# Autodesk Inventor assembly: 組合2
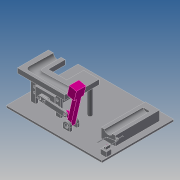
[picture p0: Inventor's stored thumbnail of the model, 180x180]
Saved by Autodesk Inventor 2015 (Build 190159000, 159)
## iProperties
Created: 2017-12-26
Part Number: 組合2
Document SubType Name: Assembly
Designer: user
Author: user
## Documents named in this file (7)
- C:\Users\user\Desktop\電腦輔助設計\組合2.iam
- C:\Users\user\Desktop\電腦輔助設計\01底板.ipt
- C:\Users\user\Desktop\電腦輔助設計\02連桿25.ipt
- C:\Users\user\Desktop\電腦輔助設計\03連桿15.ipt
- C:\Users\user\Desktop\電腦輔助設計\馬達.ipt
- C:\Users\user\Desktop\電腦輔助設計\連趕2.ipt
- C:\Users\user\Desktop\電腦輔助設計\槓桿.ipt
## Components (7 placed, 6 different names)
1. 01底板:1 — 插入:1, 貼合:1, 插入:4, 貼合:4, 角度:1, 插入:5
2. 02連桿25:1 — 插入:3, 貼合:3
3. 03連桿15:1 — 貼合:2, 插入:2, 插入:3, 角度:1
4. 馬達:1 — 插入:1, 貼合:1, 貼合:2
5. 連趕2:1 — 插入:4, 貼合:5
6. 02連桿25:2 — 插入:2, 貼合:3, 貼合:4, 貼合:5
7. 槓桿:2 — 插入:5
## Relationships (11: Insert 5, Mate 5, Angle 1)
- 插入:1 [Insert]: 01底板:1 ↔ 馬達:1
- 貼合:1 [Mate]: 01底板:1 ↔ 馬達:1
- 貼合:2 [Mate]: 03連桿15:1 ↔ 馬達:1
- 插入:2 [Insert]: 03連桿15:1 ↔ 02連桿25:2
- 插入:3 [Insert]: 02連桿25:1 ↔ 03連桿15:1
- 貼合:3 [Mate]: 02連桿25:1 ↔ 02連桿25:2
- 插入:4 [Insert]: 01底板:1 ↔ 連趕2:1
- 貼合:4 [Mate]: 01底板:1 ↔ 02連桿25:2
- 貼合:5 [Mate]: 連趕2:1 ↔ 02連桿25:2
- 角度:1 [Angle] (180 deg): 01底板:1 ↔ 03連桿15:1
- 插入:5 [Insert] (-10 mm): 01底板:1 ↔ 槓桿:2
